# Autodesk Inventor assembly: deep
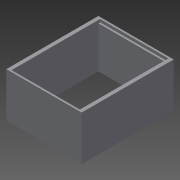
[picture p0: Inventor's stored thumbnail of the model, 180x180]
Saved by Autodesk Inventor 2014 SP1 (Build 180222100, 222)
## iProperties
Created: 2014-02-23
Part Number: deep
Document SubType Name: Assembly
Designer: Chris
Mass: 8078.57 g
Surface Area: 9997.56 cm^2
Volume: 8078.57 cm^3
Density: 1 g/cm^3
Author: Chris
## Documents named in this file (3)
- C:\Users\Chris\Documents\projects\langstroth_plain\deep\deep.iam
- C:\Users\Chris\Documents\projects\langstroth_plain\deep\deep_end.ipt
- C:\Users\Chris\Documents\projects\langstroth_plain\deep\deep_side.ipt
## Components (4 placed, 2 different names)
1. deep_end:1 — Flush:1, Flush:2, Flush:3, Flush:4, Flush:5, Flush:6
2. deep_end:2 — Flush:7, Flush:8, Flush:9, Flush:10
3. deep_side:1 — Flush:4, Flush:5, Flush:6, Flush:7, Flush:8, Flush:9, Flush:10
4. deep_side:2 — Flush:1, Flush:2, Flush:3
## Relationships (10: Flush 10)
- Flush:1: deep_end:1 ↔ deep_side:2
- Flush:2: deep_end:1 ↔ deep_side:2
- Flush:3: deep_end:1 ↔ deep_side:2
- Flush:4: deep_end:1 ↔ deep_side:1
- Flush:5: deep_end:1 ↔ deep_side:1
- Flush:6: deep_end:1 ↔ deep_side:1
- Flush:7: deep_end:2 ↔ deep_side:1
- Flush:8: deep_end:2 ↔ deep_side:1
- Flush:9: deep_end:2 ↔ deep_side:1
- Flush:10: deep_end:2 ↔ deep_side:1
